# Autodesk Inventor assembly: M178-1100
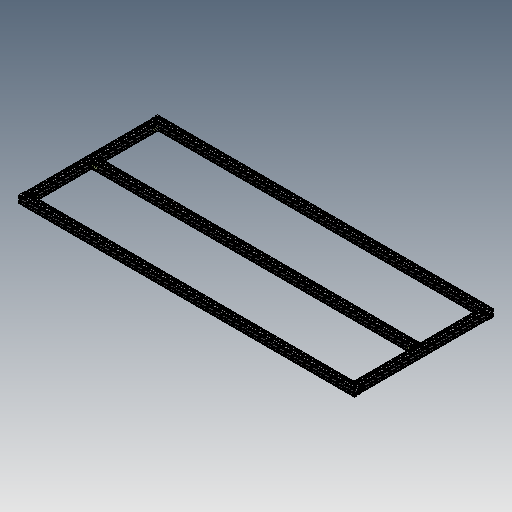
[picture p0: Inventor's stored thumbnail of the model, 512x512]
Saved by Autodesk Inventor 2018.3 (Build 223284000, 284)
## iProperties
Created: 2004-11-17
Part Number: M178-1100
Document SubType Name: Assembly
Designer: Autodesk, Inc.
Manufacturer: Standard
Standards Organization: Custom
Description: TABLE, TOP FRAM SUB ASSY
Mass: 12415.2 g
Surface Area: 32169.7 cm^2
Volume: 4521.81 cm^3
Density: 2.74563 g/cm^3
CAGE: 1LJX3
Dept. ID: Product Design
Description #2: ---
Finish #1: ---
Finish #2: ---
Material ID: ---
Project Number: ---
Author: Autodesk, Inc.
## Documents named in this file (6)
- C:\AVAInvAPI\Workspace\Test Station\Components\M178-1100.iam
- C:\AVAInvAPI\Workspace\Test Station\Components\M178-1002.ipt
- C:\AVAInvAPI\Workspace\Test Station\Components\M178-1003.ipt
- C:\AVAInvAPI\Workspace\Test Station\Components\20-004.iam
- C:\AVAInvAPI\Workspace\Test Station\Components\M178-100_Cross_Phantom.iam
- C:\Users\kelleyb.ADS\Desktop\Samples MIGRATED 2009 224 RTM_1\Standard Parts\Test Station Content\Extrusions\40 Series Profiles.ipt
## Components (9 placed, 4 different names)
1. M178-1002:1
2. M178-1002:2
3. M178-1003:3 — Flush:8
4. M178-1003:4 — Mate:4, Flush:7
5. 20-004:1 [sub-assembly]
6. 20-004:2 [sub-assembly]
7. 20-004:3 [sub-assembly]
8. 20-004:4 [sub-assembly]
9. M178-100_Cross_Phantom:1 [sub-assembly] — Mate:4, Flush:7, Flush:8
## Relationships (20: Flush 8, Mate 4, Insert 4, Angle 4)
- [Mate]: M178-1002:1 ↔ M178-1003:4
- [Flush]: M178-1002:1 ↔ M178-1003:4
- [Flush]: M178-1002:1 ↔ M178-1003:4
- [Mate]: M178-1002:1 ↔ M178-1003:3
- [Flush]: M178-1002:1 ↔ M178-1003:3
- [Flush]: M178-1002:1 ↔ M178-1003:3
- [Flush]: M178-1002:2 ↔ M178-1003:4
- [Mate]: M178-1002:2 ↔ M178-1003:4
- [Flush]: M178-1002:2 ↔ M178-1003:4
- [Insert]: M178-1003:3 ↔ 20-004:1
- [Angle] (0 deg): M178-1003:3 ↔ 20-004:1
- [Insert]: M178-1003:3 ↔ 20-004:3
- [Angle] (0 deg): M178-1003:3 ↔ 20-004:3
- [Insert]: M178-1003:4 ↔ 20-004:2
- [Angle] (0 deg): M178-1003:4 ↔ 20-004:2
- [Insert]: M178-1003:4 ↔ 20-004:4
- [Angle] (0 deg): M178-1003:4 ↔ 20-004:4
- Mate:4: M178-1003:4 ↔ M178-100_Cross_Phantom:1
- Flush:7: M178-1003:4 ↔ M178-100_Cross_Phantom:1
- Flush:8: M178-1003:3 ↔ M178-100_Cross_Phantom:1
## Named parameters: d3_d6 = 0 mm, d4_d7 = 0 mm, d5_d8 = 0 mm, d7_d12 = 0 mm, d8_d13 = 0 mm, d9_d14 = 0 mm, d10_d15 = 0 deg, d13_d16 = 0 mm
